# Autodesk Inventor assembly: Biela Completa
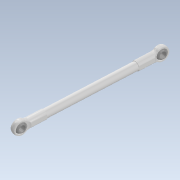
[picture p0: Inventor's stored thumbnail of the model, 180x180]
Saved by Autodesk Inventor 2021 (Build 250183000, 183)
## iProperties
Created: 2021-06-19
Part Number: Biela Completa
Document SubType Name: Assembly
Designer: Andrés Holguín
Author: Andrés Holguín
## Documents named in this file (4)
- C:\Users\andre\Documents\GitHub\Dis.-Mecatronico-E6\inventor proyecto\Motores y reductores\Biela Completa.iam
- C:\Users\andre\Documents\GitHub\Dis.-Mecatronico-E6\inventor proyecto\Motores y reductores\Eje Biela.ipt
- C:\Users\andre\Documents\GitHub\Dis.-Mecatronico-E6\inventor proyecto\Motores y reductores\soporte rotula.ipt
- C:\Users\andre\Documents\GitHub\Dis.-Mecatronico-E6\inventor proyecto\Motores y reductores\Bola Rotula.ipt
## Components (5 placed, 3 different names)
1. Eje Biela:1 — Rigid:1, Rigid:2
2. soporte rotula:2 — Rigid:1, Ball:2
3. soporte rotula:1 — Ball:1, Rigid:2
4. Bola Rotula:1 — Ball:1
5. Bola Rotula:2 — Ball:2
## Relationships (4: WeldJoint 2, BallJoint 2)
- Rigid:1 [WeldJoint]: Eje Biela:1 ↔ soporte rotula:2
- Ball:1: soporte rotula:1 ↔ Bola Rotula:1
- Rigid:2 [WeldJoint]: Eje Biela:1 ↔ soporte rotula:1
- Ball:2: soporte rotula:2 ↔ Bola Rotula:2
